# Autodesk Inventor assembly: 01-03 Zangensystem Gripper unten
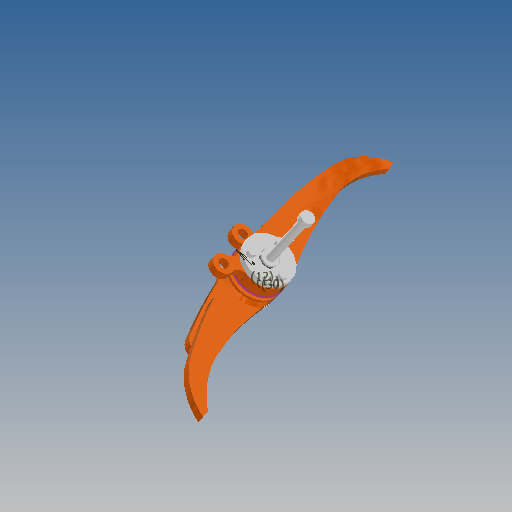
[picture p0: Inventor's stored thumbnail of the model, 512x512]
Saved by Autodesk Inventor 2026.2 (Build 302298000, 298)
## iProperties
Created: 2026-01-08
Part Number: 01-03 Zangensystem Gripper unten
Document SubType Name: Assembly
Designer: Schally
Author: Schally
## Documents named in this file (7)
- E:\06 Carologistics\02 Zeichnungen Greifer System\Gripper alt\01-03 Zangensystem Gripper unten.iam
- E:\06 Carologistics\02 Zeichnungen Greifer System\Gripper alt\01-03-03 Kugellager Tarik.ipt
- E:\06 Carologistics\02 Zeichnungen Greifer System\Gripper alt\01-03-05 Muttern.ipt
- E:\06 Carologistics\02 Zeichnungen Greifer System\Gripper alt\01-03-04 Unterlegscheibe.ipt
- E:\06 Carologistics\02 Zeichnungen Greifer System\Gripper alt\01-03-06 Schraube unten.ipt
- E:\06 Carologistics\02 Zeichnungen Greifer System\Gripper alt\01-03-01 Zange Links.iam
- E:\06 Carologistics\02 Zeichnungen Greifer System\Gripper alt\01-03-02 Zange rechts.iam
## Components (11 placed, 6 different names)
1. 01-03-03 Kugellager Tarik:1 — Passend:15, Passend:16, Passend:17, Passend:18, Passend:40, Passend:41
2. 01-03-05 Muttern:1 — Passend:15, Passend:16, Passend:37, Passend:39
3. 01-03-05 Muttern:2 — Passend:17, Passend:18, Passend:19, Passend:33
4. 01-03-05 Muttern:3 — Passend:19, Passend:21, Passend:22, Passend:34
5. 01-03-05 Muttern:4 — Passend:23, Passend:24
6. 01-03-03 Kugellager Tarik:2 — Passend:21, Passend:22, Passend:23, Passend:24, Passend:42, Passend:43
7. 01-03-04 Unterlegscheibe:1 — Passend:38, Passend:39
8. 01-03-04 Unterlegscheibe:2 — Passend:33, Passend:34
9. 01-03-06 Schraube unten:1 — Passend:37, Passend:38
10. 01-03-01 Zange Links:1 [sub-assembly] — Passend:40, Passend:41
11. 01-03-02 Zange rechts:1 [sub-assembly] — Passend:42, Passend:43
## Relationships (18: Mate 18)
- Passend:15 [Mate]: 01-03-03 Kugellager Tarik:1 ↔ 01-03-05 Muttern:1
- Passend:16 [Mate]: 01-03-03 Kugellager Tarik:1 ↔ 01-03-05 Muttern:1
- Passend:17 [Mate]: 01-03-03 Kugellager Tarik:1 ↔ 01-03-05 Muttern:2
- Passend:18 [Mate]: 01-03-03 Kugellager Tarik:1 ↔ 01-03-05 Muttern:2
- Passend:19 [Mate]: 01-03-05 Muttern:2 ↔ 01-03-05 Muttern:3
- Passend:21 [Mate]: 01-03-05 Muttern:3 ↔ 01-03-03 Kugellager Tarik:2
- Passend:22 [Mate]: 01-03-05 Muttern:3 ↔ 01-03-03 Kugellager Tarik:2
- Passend:23 [Mate]: 01-03-05 Muttern:4 ↔ 01-03-03 Kugellager Tarik:2
- Passend:24 [Mate]: 01-03-05 Muttern:4 ↔ 01-03-03 Kugellager Tarik:2
- Passend:33 [Mate]: 01-03-05 Muttern:2 ↔ 01-03-04 Unterlegscheibe:2
- Passend:34 [Mate]: 01-03-05 Muttern:3 ↔ 01-03-04 Unterlegscheibe:2
- Passend:37 [Mate]: 01-03-05 Muttern:1 ↔ 01-03-06 Schraube unten:1
- Passend:38 [Mate]: 01-03-04 Unterlegscheibe:1 ↔ 01-03-06 Schraube unten:1
- Passend:39 [Mate]: 01-03-05 Muttern:1 ↔ 01-03-04 Unterlegscheibe:1
- Passend:40 [Mate]: 01-03-03 Kugellager Tarik:1 ↔ 01-03-01 Zange Links:1
- Passend:41 [Mate]: 01-03-03 Kugellager Tarik:1 ↔ 01-03-01 Zange Links:1
- Passend:42 [Mate]: 01-03-03 Kugellager Tarik:2 ↔ 01-03-02 Zange rechts:1
- Passend:43 [Mate]: 01-03-03 Kugellager Tarik:2 ↔ 01-03-02 Zange rechts:1
